# Autodesk Inventor assembly: сборка_v1
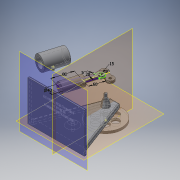
[picture p0: Inventor's stored thumbnail of the model, 180x180]
Saved by Autodesk Inventor 2017.3 (Build 213256000, 256)
## iProperties
Part Number: сборка_v1
Material: Типовые
Document SubType Name: Assembly
Designer: Alexnav
Author: Alexnav
## Documents named in this file (7)
- E:\Study\4sem\appmech\homework\1\src\5\сборка\сборка_v1.iam
- E:\Study\4sem\appmech\homework\1\src\5\cтойка\стойка_v1.ipt
- E:\Study\4sem\appmech\homework\1\src\5\кривошип\кривошип_v1.ipt
- E:\Study\4sem\appmech\homework\1\src\5\кулиса\поршень_v1.ipt
- E:\Study\4sem\appmech\homework\1\src\5\камень\стакан_v1.ipt
- E:\Study\4sem\appmech\homework\1\src\5\маховик\маховик_v1.ipt
- E:\Study\4sem\appmech\homework\1\src\5\вал\вал_v1.ipt
## Components (6 placed, 6 different names)
1. стойка_v1:1 — Совмещение:1, Совмещение:2, Совмещение:3, С поворотом:1
2. кривошип_v1:1
3. поршень_v1:1
4. стакан_v1:1
5. маховик_v1:1 — Жесткий:1
6. вал_v1:1 — С поворотом:1, Жесткий:1
## Relationships (5: Mate 3, RevoluteJoint 1, WeldJoint 1)
- Совмещение:1 [Mate]: стойка_v1:1
- Совмещение:2 [Mate]: стойка_v1:1
- Совмещение:3 [Mate]: стойка_v1:1
- С поворотом:1 [RevoluteJoint]: стойка_v1:1 ↔ вал_v1:1
- Жесткий:1 [WeldJoint]: маховик_v1:1 ↔ вал_v1:1
## Named parameters: Временная_шкала_моделирования = 0
